# Autodesk Inventor assembly: PCBPT_V3
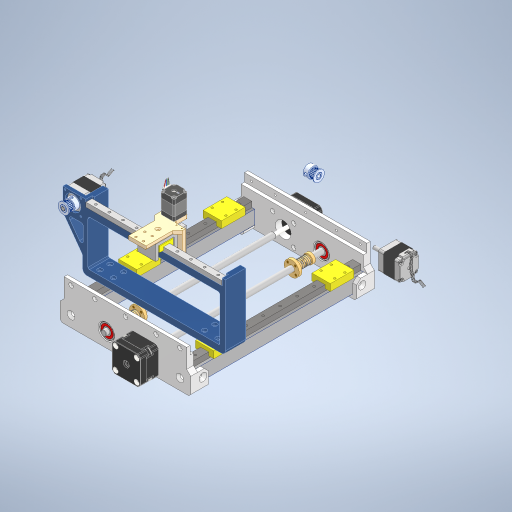
[picture p0: Inventor's stored thumbnail of the model, 512x512]
Saved by Autodesk Inventor 2024.1 (Build 281209000, 209)
## iProperties
Created: 2023-08-11
Part Number: PCBPT_V3
Document SubType Name: Assembly
Designer: l1534
Author: l1534
## Documents named in this file (21)
- C:\DATA\Documents\Lab\github\PCBPT\PCBPT_V3\Mechanical\Mechanical_1\PCBPT_V3.iam
- C:\DATA\Documents\Lab\github\PCBPT\PCBPT_V3\Mechanical\Mechanical_1\wall.ipt
- C:\DATA\Documents\Lab\github\PCBPT\PCBPT_V3\Mechanical\Mechanical_1\NEMA11\NEMA11.iam
- C:\DATA\Documents\Lab\github\PCBPT\PCBPT_V3\Mechanical\Mechanical_1\2020x260mm.ipt
- C:\DATA\Documents\Lab\github\PCBPT\PCBPT_V3\Mechanical\Mechanical_1\608-2RS Skate Board Ball Bearing\608-2RS Skate Board Ball Bearing.iam
- C:\DATA\Documents\Lab\github\PCBPT\PCBPT_V3\Mechanical\Mechanical_1\NEMA_17_PHB42S28-406A v2\NEMA_17_PHB42S28-406A v2.ipt
- C:\DATA\Documents\Lab\github\PCBPT\PCBPT_V3\Mechanical\Mechanical_1\E_box.ipt
- C:\DATA\Documents\Lab\github\PCBPT\PCBPT_V3\Mechanical\Mechanical_1\T8x250mm.ipt
- C:\DATA\Documents\Lab\github\PCBPT\PCBPT_V3\Mechanical\Mechanical_1\machine_platform.ipt
- C:\DATA\Documents\Lab\github\FlexiNet\mechanical\V1\MGN12H_rail.ipt
- C:\DATA\Documents\Lab\github\FlexiNet\mechanical\V1\MGN12C_block.ipt
- C:\DATA\Documents\Lab\github\PCBPT\PCBPT_V3\Mechanical\Mechanical_1\TR8_8(P4) Antibacklash Nut w. spring\TR8_8(P4) Antibacklash Nut w. spring.ipt
- C:\DATA\Documents\Lab\github\PCBPT\PCBPT_V3\Mechanical\Mechanical_1\probe_block_L.ipt
- C:\DATA\Documents\Lab\github\FlexiNet\mechanical\V1\MGN9x200mm_rail.ipt
- C:\DATA\Documents\Lab\github\PCBPT\PCBPT_V3\Mechanical\Mechanical_1\MGN9C_block.ipt
- C:\DATA\Documents\Lab\github\PCBPT\PCBPT_V3\Mechanical\Mechanical_1\Motor_holder_R.ipt
- C:\DATA\Documents\Lab\github\PCBPT\PCBPT_V3\Mechanical\Mechanical_1\SY20STH30-0604A\SY20STH30-0604A.ipt
- C:\DATA\Documents\Lab\github\PCBPT\PCBPT_V3\Mechanical\Mechanical_1\MGN7c_50mm_rail.ipt
- C:\DATA\Documents\Lab\github\PCBPT\PCBPT_V3\Mechanical\Mechanical_1\gantry_R.ipt
- C:\DATA\Documents\Lab\github\PCBPT\PCBPT_V3\Mechanical\Mechanical_2\GT2_motor_pulley\GT2_motor_pulley.ipt
- C:\DATA\Documents\Lab\github\PCBPT\PCBPT_V3\Mechanical\Mechanical_1\grantry_holder_R.ipt
## Components (41 placed, 20 different names)
1. wall:1 — Flush:3, Mate:7, Mate:16, Mate:17, Flush:5, Insert:2, Rigid:6, Rigid:26
2. 2020x250mm:1 — Rigid:10
3. 2020x250mm:2 — Mate:16, Mate:17, Flush:5, Mate:18, Flush:7, Rigid:11, Rigid:26
4. wall:2 — Flush:4, Mate:8, Insert:3
5. 608-2RS Skate Board Ball Bearing:2 [sub-assembly]
6. NEMA_17_PHB42S28-406A v2:1 — Flush:3, Mate:7, Rotational:1
7. NEMA_17_PHB42S28-406A v2:2 — Flush:4, Mate:8, Rotational:2
8. 608-2RS Skate Board Ball Bearing:3 [sub-assembly]
9. NEMA11:6 [sub-assembly]
10. 608-2RS Skate Board Ball Bearing:4 [sub-assembly] — Insert:2
11. 608-2RS Skate Board Ball Bearing:5 [sub-assembly] — Insert:3
12. E_box:1 — Mate:18, Flush:7
13. T8x250mm:1 — Rotational:1, Cylindrical:4
14. T8x250mm:2 — Rotational:2, Cylindrical:3
15. NEMA11:7 [sub-assembly]
16. machine_platform:1 — Rigid:6
17. MGN12H_rail:1 — Rigid:10, Slider:7, Mate:23
18. MGN12H_rail:2 — Rigid:11, Slider:9, Slider:10
19. MGN12C_block:1 — Slider:7
20. MGN12C_block:3 — Slider:9
21. MGN12C_block:4 — Slider:10, Rigid:24
22. TR8_8(P4) Antibacklash Nut w. spring:1
23. TR8_8(P4) Antibacklash Nut w. spring:2 — Rigid:17
24. TR8_8(P4) Antibacklash Nut w. spring:3 — Cylindrical:3
25. TR8_8(P4) Antibacklash Nut w. spring:4 — Cylindrical:4
26. probe_block_L:1 — Rigid:17, Rigid:20
27. MGN9x200mm_rail:1 — Rigid:25, Mate:25, Mate:26
28. MGN9C_block:1 — Mate:20, Rigid:20
29. MGN9x200mm_rail:2 — Mate:20
30. Motor_holder_R:1 — Rigid:21, Rigid:23, Rigid:29
31. SY20STH30-0604A:1 — Rigid:21
32. SY20STH30-0604A:2
33. MGN7c_50mm_rail:1 — Rigid:23
34. NEMA11:8 [sub-assembly]
35. NEMA11:9 [sub-assembly] — Rigid:27, Mate:27
36. gantry_R:2 — Rigid:24, Rigid:25, Rigid:27
37. MGN12C_block:5 — Mate:23
38. MGN9C_block:3 — Mate:25, Mate:26, Rigid:28
39. GT2_motor_pulley:1 — Mate:27
40. GT2_motor_pulley:2
41. grantry_holder_R:1 — Rigid:28, Rigid:29
## Relationships (36: WeldJoint 13, Mate 10, Flush 4, TranslationJoint 3, Insert 2, RevoluteJoint 2, CylindricalJoint 2)
- Flush:3: wall:1 ↔ NEMA_17_PHB42S28-406A v2:1
- Flush:4: wall:2 ↔ NEMA_17_PHB42S28-406A v2:2
- Mate:7: wall:1 ↔ NEMA_17_PHB42S28-406A v2:1
- Mate:8: wall:2 ↔ NEMA_17_PHB42S28-406A v2:2
- Mate:16: wall:1 ↔ 2020x250mm:2
- Mate:17: wall:1 ↔ 2020x250mm:2
- Flush:5: wall:1 ↔ 2020x250mm:2
- Insert:2: wall:1 ↔ 608-2RS Skate Board Ball Bearing:4
- Insert:3: wall:2 ↔ 608-2RS Skate Board Ball Bearing:5
- Mate:18: 2020x250mm:2 ↔ E_box:1
- Flush:7: 2020x250mm:2 ↔ E_box:1
- Rotational:1 [RevoluteJoint]: NEMA_17_PHB42S28-406A v2:1 ↔ T8x250mm:1
- Rotational:2 [RevoluteJoint]: NEMA_17_PHB42S28-406A v2:2 ↔ T8x250mm:2
- Rigid:6 [WeldJoint]: wall:1 ↔ machine_platform:1
- Rigid:10 [WeldJoint]: 2020x250mm:1 ↔ MGN12H_rail:1
- Rigid:11 [WeldJoint]: 2020x250mm:2 ↔ MGN12H_rail:2
- Slider:7 [TranslationJoint]: MGN12H_rail:1 ↔ MGN12C_block:1
- Slider:9 [TranslationJoint]: MGN12H_rail:2 ↔ MGN12C_block:3
- Slider:10 [TranslationJoint]: MGN12H_rail:2 ↔ MGN12C_block:4
- Cylindrical:3: T8x250mm:2 ↔ TR8_8(P4) Antibacklash Nut w. spring:3
- Cylindrical:4: T8x250mm:1 ↔ TR8_8(P4) Antibacklash Nut w. spring:4
- Rigid:17 [WeldJoint]: TR8_8(P4) Antibacklash Nut w. spring:2 ↔ probe_block_L:1
- Mate:20: MGN9C_block:1 ↔ MGN9x200mm_rail:2
- Rigid:20 [WeldJoint]: probe_block_L:1 ↔ MGN9C_block:1
- Rigid:21 [WeldJoint]: Motor_holder_R:1 ↔ SY20STH30-0604A:1
- Rigid:23 [WeldJoint]: Motor_holder_R:1 ↔ MGN7c_50mm_rail:1
- Rigid:24 [WeldJoint]: MGN12C_block:4 ↔ gantry_R:2
- Rigid:25 [WeldJoint]: MGN9x200mm_rail:1 ↔ gantry_R:2
- Rigid:26 [WeldJoint]: wall:1 ↔ 2020x250mm:2
- Mate:23: MGN12H_rail:1 ↔ MGN12C_block:5
- Mate:25: MGN9x200mm_rail:1 ↔ MGN9C_block:3
- Mate:26: MGN9x200mm_rail:1 ↔ MGN9C_block:3
- Rigid:27 [WeldJoint]: NEMA11:9 ↔ gantry_R:2
- Mate:27: NEMA11:9 ↔ GT2_motor_pulley:1
- Rigid:28 [WeldJoint]: MGN9C_block:3 ↔ grantry_holder_R:1
- Rigid:29 [WeldJoint]: Motor_holder_R:1 ↔ grantry_holder_R:1
